# Autodesk Inventor assembly: MaleHeaderPin_1x6_90
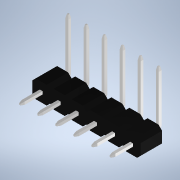
[picture p0: Inventor's stored thumbnail of the model, 180x180]
Saved by Autodesk Inventor 2021 (Build 250183000, 183)
## iProperties
Created: 2021-07-24
Part Number: MaleHeaderPin_1x6_90
Document SubType Name: Assembly
Designer: ermoz
Author: ermoz
## Documents named in this file (2)
- D:\Moje Wyczyny\My_Poor_Projects\Sneak100_MiniSumo\minisumo-sneak100\mechanics\ElectricElements\MaleHeaderPin_1x6_90.iam
- D:\Moje Wyczyny\My_Poor_Projects\Sneak100_MiniSumo\minisumo-sneak100\mechanics\ElectricElements\MaleHeaderPin_90.ipt
## Components (6 placed, 1 different names)
1. MaleHeaderPin_90:1 — Mate:1, Flush:1, Flush:6
2. MaleHeaderPin_90:2 — Mate:1, Mate:2, Flush:1, Flush:2, Flush:6, Flush:7
3. MaleHeaderPin_90:3 — Mate:2, Mate:3, Flush:2, Flush:3, Flush:7, Flush:8
4. MaleHeaderPin_90:4 — Mate:3, Mate:4, Flush:3, Flush:4, Flush:8, Flush:9
5. MaleHeaderPin_90:5 — Mate:4, Mate:5, Flush:4, Flush:5, Flush:9, Flush:10
6. MaleHeaderPin_90:6 — Mate:5, Flush:5, Flush:10
## Relationships (15: Flush 10, Mate 5)
- Mate:1: MaleHeaderPin_90:1 ↔ MaleHeaderPin_90:2
- Mate:2: MaleHeaderPin_90:2 ↔ MaleHeaderPin_90:3
- Mate:3: MaleHeaderPin_90:3 ↔ MaleHeaderPin_90:4
- Mate:4: MaleHeaderPin_90:4 ↔ MaleHeaderPin_90:5
- Mate:5: MaleHeaderPin_90:5 ↔ MaleHeaderPin_90:6
- Flush:1: MaleHeaderPin_90:1 ↔ MaleHeaderPin_90:2
- Flush:2: MaleHeaderPin_90:2 ↔ MaleHeaderPin_90:3
- Flush:3: MaleHeaderPin_90:3 ↔ MaleHeaderPin_90:4
- Flush:4: MaleHeaderPin_90:4 ↔ MaleHeaderPin_90:5
- Flush:5: MaleHeaderPin_90:5 ↔ MaleHeaderPin_90:6
- Flush:6: MaleHeaderPin_90:1 ↔ MaleHeaderPin_90:2
- Flush:7: MaleHeaderPin_90:2 ↔ MaleHeaderPin_90:3
- Flush:8: MaleHeaderPin_90:3 ↔ MaleHeaderPin_90:4
- Flush:9: MaleHeaderPin_90:4 ↔ MaleHeaderPin_90:5
- Flush:10: MaleHeaderPin_90:5 ↔ MaleHeaderPin_90:6
